# Autodesk Inventor assembly: Frame
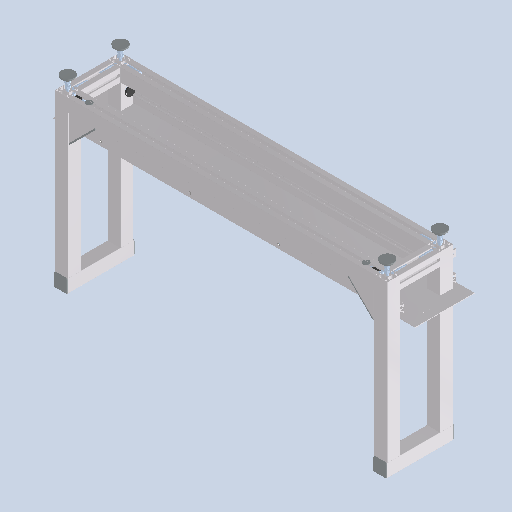
[picture p0: Inventor's stored thumbnail of the model, 512x512]
Saved by Autodesk Inventor 2025 (Build 290162010, 162A)
## iProperties
Created: 2025-01-18
Part Number: Frame
Document SubType Name: Assembly
Designer: Admin
Author: Admin
## Documents named in this file (26)
- C:\Users\Admin\GIT\HDVKBM\CAD\Krandemonstrator\Frame.iam
- C:\Users\Admin\GIT\HDVKBM\CAD\Krandemonstrator\item_61193_profil-x-8-40x40-2no180-_930_high\item_61193_profil-x-8-40x40-2no180-_930_high.ipt
- C:\Users\Admin\GIT\HDVKBM\CAD\Krandemonstrator\item_49291_profil-x-8-40x40-leicht-_120_high\item_49291_profil-x-8-40x40-leicht-_120_high.ipt
- C:\Users\Admin\GIT\HDVKBM\CAD\Krandemonstrator\item_49288_profil-x-8-40x40-4no-lei_200_high\item_49288_profil-x-8-40x40-4no-lei_200_high.ipt
- C:\Users\Admin\GIT\HDVKBM\CAD\Krandemonstrator\item_49288_profil-x-8-40x40-4no-lei_475_high\item_49288_profil-x-8-40x40-4no-lei_475_high.ipt
- C:\Users\Admin\GIT\HDVKBM\CAD\Krandemonstrator\item_67284_automatik-verbindungssat__high\item_67284_automatik-verbindungssat__high.ipt
- C:\Users\Admin\GIT\HDVKBM\CAD\Krandemonstrator\item_63697_stellfuss-d40-m8x60-grau_35_0_high\item_63697_stellfuss-d40-m8x60-grau_35_0_high.ipt
- C:\Users\Admin\GIT\HDVKBM\CAD\Krandemonstrator\item_62716_abdeckkappe-8-40x40-grau__high\item_62716_abdeckkappe-8-40x40-grau__high.ipt
- C:\Users\Admin\GIT\HDVKBM\CAD\Krandemonstrator\item_48996_automatik-verbindungssat__high\item_48996_automatik-verbindungssat__high.ipt
- C:\Users\Admin\GIT\HDVKBM\CAD\Krandemonstrator\item_41123_winkel-8-80x80-zn-weissa__high\item_41123_winkel-8-80x80-zn-weissa__high.ipt
- C:\Users\Admin\GIT\HDVKBM\CAD\Krandemonstrator\item_2618_nutenstein-8-st-m8-verzi__high\item_2618_nutenstein-8-st-m8-verzi__high.ipt
- C:\Users\Admin\Documents\Inventor\Content Center Files\R2025\de-DE\AS 1420\AS 1420 - 1973 - M8 x 16.ipt
- C:\Users\Admin\GIT\HDVKBM\CAD\Krandemonstrator\item_62758_winkel-abdeckkappe-8-80x__high\item_62758_winkel-abdeckkappe-8-80x__high.ipt
- C:\Users\Admin\GIT\HDVKBM\CAD\Krandemonstrator\item_43452_stellfuss-d30-m6x45-schw_20_0_high\item_43452_stellfuss-d30-m6x45-schw_20_0_high.ipt
- C:\Users\Admin\GIT\HDVKBM\CAD\Krandemonstrator\item_2623_nutenstein-8-st-m6-verzi__high\item_2623_nutenstein-8-st-m6-verzi__high.ipt
- C:\Users\Admin\GIT\HDVKBM\CAD\Krandemonstrator\item_42005_nutenstein-8-st-m5-verzi__high\item_42005_nutenstein-8-st-m5-verzi__high.ipt
- C:\Users\Admin\GIT\HDVKBM\CAD\Krandemonstrator\item_67777_winkel-5-20-weissalumini__high\item_67777_winkel-5-20-weissalumini__high.ipt
- C:\Users\Admin\GIT\HDVKBM\CAD\Krandemonstrator\item_68092_befestigungssatz-5-2-4mm_2_high\item_68092_befestigungssatz-5-2-4mm_2_high.ipt
- C:\Users\Admin\Documents\Inventor\Content Center Files\R2025\de-DE\DIN 7991(2)\DIN 7991 - M5x12.ipt
- C:\Users\Admin\GIT\HDVKBM\CAD\Krandemonstrator\item_37003_profil-5-20x20-natur-370_990_high\item_37003_profil-5-20x20-natur-370_990_high.ipt
- C:\Users\Admin\GIT\HDVKBM\CAD\Krandemonstrator\item_43767_profil-5-20x20-2n180-nat_990_high\item_43767_profil-5-20x20-2n180-nat_990_high.ipt
- C:\Users\Admin\GIT\HDVKBM\CAD\Krandemonstrator\item_47308_blech-al-2mm-naturfarben_990_90_high\item_47308_blech-al-2mm-naturfarben_990_90_high.ipt
- C:\Users\Admin\GIT\HDVKBM\CAD\Krandemonstrator\item_47308_blech-al-2mm-naturfarben_1100_180_high\item_47308_blech-al-2mm-naturfarben_1100_180_high.ipt
- C:\Users\Admin\Documents\Inventor\Content Center Files\R2025\de-DE\DIN 7991(2)\DIN 7991 - M5x16.ipt
- C:\Users\Admin\Documents\Inventor\Content Center Files\R2025\de-DE\DIN 7991(2)\DIN 7991 - M4x8.ipt
- C:\Users\Admin\GIT\HDVKBM\CAD\Krandemonstrator\item_37006_nutenstein-5-st-m4-verzi__high\item_37006_nutenstein-5-st-m4-verzi__high.ipt
## Components (88 placed, 25 different names)
1. item_61193_profil-x-8-40x40-2no180-_930_high:1 — Starr:12, Starr:13, Starr:14
2. item_61193_profil-x-8-40x40-2no180-_930_high:2 — Starr:17, Starr:27, Planar:1, Planar:2, Starr:47, Starr:48, Planar:68
3. item_49291_profil-x-8-40x40-leicht-_120_high:1 — Starr:7, Starr:8, Starr:9
4. item_49291_profil-x-8-40x40-leicht-_120_high:2 — Starr:24, Starr:25, Starr:26
5. item_49288_profil-x-8-40x40-4no-lei_200_high:1 — Starr:18, Starr:19, Starr:21, Starr:23
6. item_49288_profil-x-8-40x40-4no-lei_200_high:2 — Starr:2, Starr:4, Starr:5, Starr:6
7. item_49288_profil-x-8-40x40-4no-lei_475_high:1 — Starr:20, Starr:21, Starr:28, Starr:41, Verschiebbar:6, Verschiebbar:7, Planar:60
8. item_49288_profil-x-8-40x40-4no-lei_475_high:2 — Starr:22, Starr:23, Starr:25, Starr:27, Starr:29, Verschiebbar:2, Verschiebbar:4
9. item_49288_profil-x-8-40x40-4no-lei_475_high:3 — Starr:3, Starr:4, Starr:11, Starr:17, Verschiebbar:1, Verschiebbar:3, Planar:66
10. item_49288_profil-x-8-40x40-4no-lei_475_high:4 — Starr:1, Starr:2, Starr:9, Starr:10, Starr:14, Starr:43, Verschiebbar:5, Verschiebbar:8
11. item_67284_automatik-verbindungssat__high:1 — Starr:1
12. item_67284_automatik-verbindungssat__high:2 — Starr:20
13. item_67284_automatik-verbindungssat__high:3 — Starr:3
14. item_67284_automatik-verbindungssat__high:4 — Starr:24
15. item_67284_automatik-verbindungssat__high:5 — Starr:12
16. item_67284_automatik-verbindungssat__high:6 — Starr:13
17. item_67284_automatik-verbindungssat__high:7 — Starr:8
18. item_67284_automatik-verbindungssat__high:8 — Starr:7
19. item_48996_automatik-verbindungssat__high:1 — Starr:47
20. item_48996_automatik-verbindungssat__high:2 — Starr:48
21. item_67284_automatik-verbindungssat__high:11 — Starr:22
22. item_67284_automatik-verbindungssat__high:12 — Starr:26
23. item_63697_stellfuss-d40-m8x60-grau_35_0_high:1 — Starr:10
24. item_63697_stellfuss-d40-m8x60-grau_35_0_high:2 — Starr:11
25. item_63697_stellfuss-d40-m8x60-grau_35_0_high:3 — Starr:28
26. item_63697_stellfuss-d40-m8x60-grau_35_0_high:4 — Starr:29
27. item_62716_abdeckkappe-8-40x40-grau__high:1 — Starr:5
28. item_62716_abdeckkappe-8-40x40-grau__high:2 — Starr:6
29. item_62716_abdeckkappe-8-40x40-grau__high:3 — Starr:18
30. item_62716_abdeckkappe-8-40x40-grau__high:4 — Starr:19
31. item_41123_winkel-8-80x80-zn-weissa__high:1 — Einfügen:3, Einfügen:4, Einfügen:7, Einfügen:8, Verschiebbar:2, Planar:2, Starr:38
32. item_41123_winkel-8-80x80-zn-weissa__high:2 — Einfügen:1, Einfügen:2, Einfügen:5, Einfügen:6, Verschiebbar:1, Planar:1, Starr:39
33. item_2618_nutenstein-8-st-m8-verzi__high:1 — Starr:34
34. item_2618_nutenstein-8-st-m8-verzi__high:2 — Starr:31
35. item_2618_nutenstein-8-st-m8-verzi__high:3 — Starr:36
36. item_2618_nutenstein-8-st-m8-verzi__high:4 — Starr:32
37. item_2618_nutenstein-8-st-m8-verzi__high:5 — Starr:37
38. item_2618_nutenstein-8-st-m8-verzi__high:6 — Starr:30
39. item_2618_nutenstein-8-st-m8-verzi__high:7 — Starr:35
40. item_2618_nutenstein-8-st-m8-verzi__high:8 — Starr:33
41. AS 1420 - Metrisch M8 x 16:1 — Einfügen:1, Starr:37
42. AS 1420 - Metrisch M8 x 16:2 — Einfügen:2, Starr:36
43. AS 1420 - Metrisch M8 x 16:3 — Einfügen:3, Starr:35
44. AS 1420 - Metrisch M8 x 16:4 — Einfügen:4, Starr:34
45. AS 1420 - Metrisch M8 x 16:5 — Einfügen:5, Starr:31
46. AS 1420 - Metrisch M8 x 16:6 — Einfügen:6, Starr:30
47. AS 1420 - Metrisch M8 x 16:7 — Einfügen:7, Starr:33
48. AS 1420 - Metrisch M8 x 16:8 — Einfügen:8, Starr:32
49. item_62758_winkel-abdeckkappe-8-80x__high:1 — Starr:38
50. item_62758_winkel-abdeckkappe-8-80x__high:2 — Starr:39
51. item_43452_stellfuss-d30-m6x45-schw_20_0_high:1 — Starr:40
52. item_43452_stellfuss-d30-m6x45-schw_20_0_high:2 — Starr:42
53. item_2623_nutenstein-8-st-m6-verzi__high:1 — Starr:40, Starr:41
54. item_2623_nutenstein-8-st-m6-verzi__high:2 — Starr:42, Starr:43
55. item_42005_nutenstein-8-st-m5-verzi__high:1 — Starr:45
56. item_42005_nutenstein-8-st-m5-verzi__high:2 — Starr:44
57. item_42005_nutenstein-8-st-m5-verzi__high:3 — Starr:52
58. item_42005_nutenstein-8-st-m5-verzi__high:4 — Starr:53
59. item_67777_winkel-5-20-weissalumini__high:1 — Starr:44, Starr:49, Passend:1, Verschiebbar:6, Planar:59, Planar:61
60. item_67777_winkel-5-20-weissalumini__high:2 — Starr:45, Starr:46, Passend:2, Verschiebbar:5, Planar:62
61. item_67777_winkel-5-20-weissalumini__high:3 — Starr:50, Passend:3, Starr:53, Verschiebbar:4
62. item_67777_winkel-5-20-weissalumini__high:4 — Starr:51, Passend:4, Starr:52, Verschiebbar:3, Planar:67
63. item_68092_befestigungssatz-5-2-4mm_2_high:1 — Starr:49
64. item_68092_befestigungssatz-5-2-4mm_2_high:2 — Starr:46
65. item_68092_befestigungssatz-5-2-4mm_2_high:3 — Starr:50
66. item_68092_befestigungssatz-5-2-4mm_2_high:4 — Starr:51
67. DIN 7991 M5x12:1 — Passend:1
68. DIN 7991 M5x12:2 — Passend:2
69. DIN 7991 M5x16:2 — Passend:3
70. DIN 7991 M5x16:1 — Passend:4
71. item_37003_profil-5-20x20-natur-370_990_high:1 — Planar:12, Planar:64
72. item_43767_profil-5-20x20-2n180-nat_990_high:1 — Planar:59, Planar:60, Planar:61, Planar:62, Planar:63
73. item_67777_winkel-5-20-weissalumini__high:5 — Verschiebbar:7, Starr:55, Starr:56
74. item_67777_winkel-5-20-weissalumini__high:6 — Verschiebbar:8, Starr:54, Starr:57
75. item_42005_nutenstein-8-st-m5-verzi__high:5 — Starr:54
76. item_42005_nutenstein-8-st-m5-verzi__high:6 — Starr:55
77. DIN 7991 M5x12:5 — Starr:56
78. DIN 7991 M5x12:6 — Starr:57
79. item_47308_blech-al-2mm-naturfarben_990_90_high:1 — Planar:64, Planar:65, Planar:66, Planar:13, Planar:67, Drehbar:1, Drehbar:2, Starr:58, Starr:59, Verschiebbar:9
80. item_47308_blech-al-2mm-naturfarben_1100_180_high:1 — Planar:12, Planar:13, Planar:63, Planar:65, Verschiebbar:9, Planar:68
81. DIN 7991 M4x8:1 — Starr:59, Starr:60
82. DIN 7991 M4x8:2 — Drehbar:2, Starr:62
83. DIN 7991 M4x8:3 — Drehbar:1, Starr:61
84. DIN 7991 M4x8:4 — Starr:58, Starr:63
85. item_37006_nutenstein-5-st-m4-verzi__high:1 — Starr:61
86. item_37006_nutenstein-5-st-m4-verzi__high:2 — Starr:63
87. item_37006_nutenstein-5-st-m4-verzi__high:3 — Starr:62
88. item_37006_nutenstein-5-st-m4-verzi__high:4 — Starr:60
## Relationships (101: WeldJoint 61, PlanarJoint 17, TranslationJoint 9, Insert 8, Mate 4, RevoluteJoint 2)
- Starr:1 [WeldJoint]: item_49288_profil-x-8-40x40-4no-lei_475_high:4 ↔ item_67284_automatik-verbindungssat__high:1
- Starr:2 [WeldJoint]: item_49288_profil-x-8-40x40-4no-lei_200_high:2 ↔ item_49288_profil-x-8-40x40-4no-lei_475_high:4
- Starr:3 [WeldJoint]: item_49288_profil-x-8-40x40-4no-lei_475_high:3 ↔ item_67284_automatik-verbindungssat__high:3
- Starr:4 [WeldJoint]: item_49288_profil-x-8-40x40-4no-lei_200_high:2 ↔ item_49288_profil-x-8-40x40-4no-lei_475_high:3
- Starr:5 [WeldJoint]: item_49288_profil-x-8-40x40-4no-lei_200_high:2 ↔ item_62716_abdeckkappe-8-40x40-grau__high:1
- Starr:6 [WeldJoint]: item_49288_profil-x-8-40x40-4no-lei_200_high:2 ↔ item_62716_abdeckkappe-8-40x40-grau__high:2
- Starr:7 [WeldJoint]: item_49291_profil-x-8-40x40-leicht-_120_high:1 ↔ item_67284_automatik-verbindungssat__high:8
- Starr:8 [WeldJoint]: item_49291_profil-x-8-40x40-leicht-_120_high:1 ↔ item_67284_automatik-verbindungssat__high:7
- Starr:9 [WeldJoint]: item_49291_profil-x-8-40x40-leicht-_120_high:1 ↔ item_49288_profil-x-8-40x40-4no-lei_475_high:4
- Starr:10 [WeldJoint]: item_49288_profil-x-8-40x40-4no-lei_475_high:4 ↔ item_63697_stellfuss-d40-m8x60-grau_35_0_high:1
- Starr:11 [WeldJoint]: item_49288_profil-x-8-40x40-4no-lei_475_high:3 ↔ item_63697_stellfuss-d40-m8x60-grau_35_0_high:2
- Starr:12 [WeldJoint]: item_61193_profil-x-8-40x40-2no180-_930_high:1 ↔ item_67284_automatik-verbindungssat__high:5
- Starr:13 [WeldJoint]: item_61193_profil-x-8-40x40-2no180-_930_high:1 ↔ item_67284_automatik-verbindungssat__high:6
- Starr:14 [WeldJoint]: item_61193_profil-x-8-40x40-2no180-_930_high:1 ↔ item_49288_profil-x-8-40x40-4no-lei_475_high:4
- Starr:17 [WeldJoint]: item_61193_profil-x-8-40x40-2no180-_930_high:2 ↔ item_49288_profil-x-8-40x40-4no-lei_475_high:3
- Starr:18 [WeldJoint]: item_49288_profil-x-8-40x40-4no-lei_200_high:1 ↔ item_62716_abdeckkappe-8-40x40-grau__high:3
- Starr:19 [WeldJoint]: item_49288_profil-x-8-40x40-4no-lei_200_high:1 ↔ item_62716_abdeckkappe-8-40x40-grau__high:4
- Starr:20 [WeldJoint]: item_49288_profil-x-8-40x40-4no-lei_475_high:1 ↔ item_67284_automatik-verbindungssat__high:2
- Starr:21 [WeldJoint]: item_49288_profil-x-8-40x40-4no-lei_200_high:1 ↔ item_49288_profil-x-8-40x40-4no-lei_475_high:1
- Starr:22 [WeldJoint]: item_49288_profil-x-8-40x40-4no-lei_475_high:2 ↔ item_67284_automatik-verbindungssat__high:11
- Starr:23 [WeldJoint]: item_49288_profil-x-8-40x40-4no-lei_200_high:1 ↔ item_49288_profil-x-8-40x40-4no-lei_475_high:2
- Starr:24 [WeldJoint]: item_49291_profil-x-8-40x40-leicht-_120_high:2 ↔ item_67284_automatik-verbindungssat__high:4
- Starr:25 [WeldJoint]: item_49291_profil-x-8-40x40-leicht-_120_high:2 ↔ item_49288_profil-x-8-40x40-4no-lei_475_high:2
- Starr:26 [WeldJoint]: item_49291_profil-x-8-40x40-leicht-_120_high:2 ↔ item_67284_automatik-verbindungssat__high:12
- Starr:27 [WeldJoint]: item_61193_profil-x-8-40x40-2no180-_930_high:2 ↔ item_49288_profil-x-8-40x40-4no-lei_475_high:2
- Starr:28 [WeldJoint]: item_49288_profil-x-8-40x40-4no-lei_475_high:1 ↔ item_63697_stellfuss-d40-m8x60-grau_35_0_high:3
- Starr:29 [WeldJoint]: item_49288_profil-x-8-40x40-4no-lei_475_high:2 ↔ item_63697_stellfuss-d40-m8x60-grau_35_0_high:4
- Einfügen:1 [Insert]: item_41123_winkel-8-80x80-zn-weissa__high:2 ↔ AS 1420 - Metrisch M8 x 16:1
- Einfügen:2 [Insert]: item_41123_winkel-8-80x80-zn-weissa__high:2 ↔ AS 1420 - Metrisch M8 x 16:2
- Einfügen:3 [Insert]: item_41123_winkel-8-80x80-zn-weissa__high:1 ↔ AS 1420 - Metrisch M8 x 16:3
- Einfügen:4 [Insert]: item_41123_winkel-8-80x80-zn-weissa__high:1 ↔ AS 1420 - Metrisch M8 x 16:4
- Einfügen:5 [Insert]: item_41123_winkel-8-80x80-zn-weissa__high:2 ↔ AS 1420 - Metrisch M8 x 16:5
- Einfügen:6 [Insert]: item_41123_winkel-8-80x80-zn-weissa__high:2 ↔ AS 1420 - Metrisch M8 x 16:6
- Einfügen:7 [Insert]: item_41123_winkel-8-80x80-zn-weissa__high:1 ↔ AS 1420 - Metrisch M8 x 16:7
- Einfügen:8 [Insert]: item_41123_winkel-8-80x80-zn-weissa__high:1 ↔ AS 1420 - Metrisch M8 x 16:8
- Starr:30 [WeldJoint]: item_2618_nutenstein-8-st-m8-verzi__high:6 ↔ AS 1420 - Metrisch M8 x 16:6
- Starr:31 [WeldJoint]: item_2618_nutenstein-8-st-m8-verzi__high:2 ↔ AS 1420 - Metrisch M8 x 16:5
- Starr:32 [WeldJoint]: item_2618_nutenstein-8-st-m8-verzi__high:4 ↔ AS 1420 - Metrisch M8 x 16:8
- Starr:33 [WeldJoint]: item_2618_nutenstein-8-st-m8-verzi__high:8 ↔ AS 1420 - Metrisch M8 x 16:7
- Starr:34 [WeldJoint]: item_2618_nutenstein-8-st-m8-verzi__high:1 ↔ AS 1420 - Metrisch M8 x 16:4
- Starr:35 [WeldJoint]: item_2618_nutenstein-8-st-m8-verzi__high:7 ↔ AS 1420 - Metrisch M8 x 16:3
- Starr:36 [WeldJoint]: item_2618_nutenstein-8-st-m8-verzi__high:3 ↔ AS 1420 - Metrisch M8 x 16:2
- Starr:37 [WeldJoint]: item_2618_nutenstein-8-st-m8-verzi__high:5 ↔ AS 1420 - Metrisch M8 x 16:1
- Verschiebbar:1 [TranslationJoint]: item_49288_profil-x-8-40x40-4no-lei_475_high:3 ↔ item_41123_winkel-8-80x80-zn-weissa__high:2
- Planar:1: item_61193_profil-x-8-40x40-2no180-_930_high:2 ↔ item_41123_winkel-8-80x80-zn-weissa__high:2
- Verschiebbar:2 [TranslationJoint]: item_49288_profil-x-8-40x40-4no-lei_475_high:2 ↔ item_41123_winkel-8-80x80-zn-weissa__high:1
- Planar:2: item_61193_profil-x-8-40x40-2no180-_930_high:2 ↔ item_41123_winkel-8-80x80-zn-weissa__high:1
- Starr:38 [WeldJoint]: item_41123_winkel-8-80x80-zn-weissa__high:1 ↔ item_62758_winkel-abdeckkappe-8-80x__high:1
- Starr:39 [WeldJoint]: item_41123_winkel-8-80x80-zn-weissa__high:2 ↔ item_62758_winkel-abdeckkappe-8-80x__high:2
- Starr:40 [WeldJoint]: item_43452_stellfuss-d30-m6x45-schw_20_0_high:1 ↔ item_2623_nutenstein-8-st-m6-verzi__high:1
- Starr:41 [WeldJoint] (-60 mm): item_49288_profil-x-8-40x40-4no-lei_475_high:1 ↔ item_2623_nutenstein-8-st-m6-verzi__high:1
- Starr:42 [WeldJoint]: item_43452_stellfuss-d30-m6x45-schw_20_0_high:2 ↔ item_2623_nutenstein-8-st-m6-verzi__high:2
- Starr:43 [WeldJoint] (-60 mm): item_49288_profil-x-8-40x40-4no-lei_475_high:4 ↔ item_2623_nutenstein-8-st-m6-verzi__high:2
- Starr:44 [WeldJoint] (-5 mm): item_42005_nutenstein-8-st-m5-verzi__high:2 ↔ item_67777_winkel-5-20-weissalumini__high:1
- Starr:45 [WeldJoint] (-5 mm): item_42005_nutenstein-8-st-m5-verzi__high:1 ↔ item_67777_winkel-5-20-weissalumini__high:2
- Starr:46 [WeldJoint]: item_67777_winkel-5-20-weissalumini__high:2 ↔ item_68092_befestigungssatz-5-2-4mm_2_high:2
- Starr:47 [WeldJoint]: item_61193_profil-x-8-40x40-2no180-_930_high:2 ↔ item_48996_automatik-verbindungssat__high:1
- Starr:48 [WeldJoint]: item_61193_profil-x-8-40x40-2no180-_930_high:2 ↔ item_48996_automatik-verbindungssat__high:2
- Starr:49 [WeldJoint]: item_67777_winkel-5-20-weissalumini__high:1 ↔ item_68092_befestigungssatz-5-2-4mm_2_high:1
- Passend:1 [Mate]: item_67777_winkel-5-20-weissalumini__high:1 ↔ DIN 7991 M5x12:1
- Passend:2 [Mate]: item_67777_winkel-5-20-weissalumini__high:2 ↔ DIN 7991 M5x12:2
- Starr:50 [WeldJoint]: item_67777_winkel-5-20-weissalumini__high:3 ↔ item_68092_befestigungssatz-5-2-4mm_2_high:3
- Starr:51 [WeldJoint]: item_67777_winkel-5-20-weissalumini__high:4 ↔ item_68092_befestigungssatz-5-2-4mm_2_high:4
- Passend:3 [Mate]: item_67777_winkel-5-20-weissalumini__high:3 ↔ DIN 7991 M5x16:2
- Passend:4 [Mate]: item_67777_winkel-5-20-weissalumini__high:4 ↔ DIN 7991 M5x16:1
- Starr:52 [WeldJoint] (-5 mm): item_42005_nutenstein-8-st-m5-verzi__high:3 ↔ item_67777_winkel-5-20-weissalumini__high:4
- Starr:53 [WeldJoint] (-5 mm): item_42005_nutenstein-8-st-m5-verzi__high:4 ↔ item_67777_winkel-5-20-weissalumini__high:3
- Verschiebbar:3 [TranslationJoint] (2 mm): item_49288_profil-x-8-40x40-4no-lei_475_high:3 ↔ item_67777_winkel-5-20-weissalumini__high:4
- Verschiebbar:4 [TranslationJoint]: item_49288_profil-x-8-40x40-4no-lei_475_high:2 ↔ item_67777_winkel-5-20-weissalumini__high:3
- [PlanarJoint]: item_67777_winkel-5-20-weissalumini__high:4 ↔ item_37003_profil-5-20x20-natur-370_990_high:1
- [PlanarJoint]: item_67777_winkel-5-20-weissalumini__high:4 ↔ item_37003_profil-5-20x20-natur-370_990_high:1
- [PlanarJoint]: item_67777_winkel-5-20-weissalumini__high:3 ↔ item_37003_profil-5-20x20-natur-370_990_high:1
- Verschiebbar:5 [TranslationJoint]: item_49288_profil-x-8-40x40-4no-lei_475_high:4 ↔ item_67777_winkel-5-20-weissalumini__high:2
- Verschiebbar:6 [TranslationJoint]: item_49288_profil-x-8-40x40-4no-lei_475_high:1 ↔ item_67777_winkel-5-20-weissalumini__high:1
- Verschiebbar:7 [TranslationJoint]: item_49288_profil-x-8-40x40-4no-lei_475_high:1 ↔ item_67777_winkel-5-20-weissalumini__high:5
- Verschiebbar:8 [TranslationJoint]: item_49288_profil-x-8-40x40-4no-lei_475_high:4 ↔ item_67777_winkel-5-20-weissalumini__high:6
- Starr:54 [WeldJoint] (5 mm): item_67777_winkel-5-20-weissalumini__high:6 ↔ item_42005_nutenstein-8-st-m5-verzi__high:5
- Starr:55 [WeldJoint] (5 mm): item_67777_winkel-5-20-weissalumini__high:5 ↔ item_42005_nutenstein-8-st-m5-verzi__high:6
- Starr:56 [WeldJoint]: item_67777_winkel-5-20-weissalumini__high:5 ↔ DIN 7991 M5x12:5
- Starr:57 [WeldJoint]: item_67777_winkel-5-20-weissalumini__high:6 ↔ DIN 7991 M5x12:6
- Planar:12: item_37003_profil-5-20x20-natur-370_990_high:1 ↔ item_47308_blech-al-2mm-naturfarben_1100_180_high:1
- Planar:13: item_47308_blech-al-2mm-naturfarben_990_90_high:1 ↔ item_47308_blech-al-2mm-naturfarben_1100_180_high:1
- Planar:59: item_67777_winkel-5-20-weissalumini__high:1 ↔ item_43767_profil-5-20x20-2n180-nat_990_high:1
- Planar:60: item_49288_profil-x-8-40x40-4no-lei_475_high:1 ↔ item_43767_profil-5-20x20-2n180-nat_990_high:1
- Planar:61: item_67777_winkel-5-20-weissalumini__high:1 ↔ item_43767_profil-5-20x20-2n180-nat_990_high:1
- Planar:62: item_67777_winkel-5-20-weissalumini__high:2 ↔ item_43767_profil-5-20x20-2n180-nat_990_high:1
- Planar:63: item_43767_profil-5-20x20-2n180-nat_990_high:1 ↔ item_47308_blech-al-2mm-naturfarben_1100_180_high:1
- Planar:64: item_37003_profil-5-20x20-natur-370_990_high:1 ↔ item_47308_blech-al-2mm-naturfarben_990_90_high:1
- Planar:65: item_47308_blech-al-2mm-naturfarben_990_90_high:1 ↔ item_47308_blech-al-2mm-naturfarben_1100_180_high:1
- Planar:66: item_49288_profil-x-8-40x40-4no-lei_475_high:3 ↔ item_47308_blech-al-2mm-naturfarben_990_90_high:1
- Planar:67: item_67777_winkel-5-20-weissalumini__high:4 ↔ item_47308_blech-al-2mm-naturfarben_990_90_high:1
- Drehbar:1 [RevoluteJoint]: item_47308_blech-al-2mm-naturfarben_990_90_high:1 ↔ DIN 7991 M4x8:3
- Drehbar:2 [RevoluteJoint]: item_47308_blech-al-2mm-naturfarben_990_90_high:1 ↔ DIN 7991 M4x8:2
- Starr:58 [WeldJoint]: item_47308_blech-al-2mm-naturfarben_990_90_high:1 ↔ DIN 7991 M4x8:4
- Starr:59 [WeldJoint]: item_47308_blech-al-2mm-naturfarben_990_90_high:1 ↔ DIN 7991 M4x8:1
- Starr:60 [WeldJoint]: DIN 7991 M4x8:1 ↔ item_37006_nutenstein-5-st-m4-verzi__high:4
- Starr:61 [WeldJoint]: DIN 7991 M4x8:3 ↔ item_37006_nutenstein-5-st-m4-verzi__high:1
- Starr:62 [WeldJoint]: DIN 7991 M4x8:2 ↔ item_37006_nutenstein-5-st-m4-verzi__high:3
- Starr:63 [WeldJoint]: DIN 7991 M4x8:4 ↔ item_37006_nutenstein-5-st-m4-verzi__high:2
- Verschiebbar:9 [TranslationJoint]: item_47308_blech-al-2mm-naturfarben_990_90_high:1 ↔ item_47308_blech-al-2mm-naturfarben_1100_180_high:1
- Planar:68 (75 mm): item_61193_profil-x-8-40x40-2no180-_930_high:2 ↔ item_47308_blech-al-2mm-naturfarben_1100_180_high:1
